# Autodesk Inventor assembly: 3.25'' Traction Wheel, Square Insert2
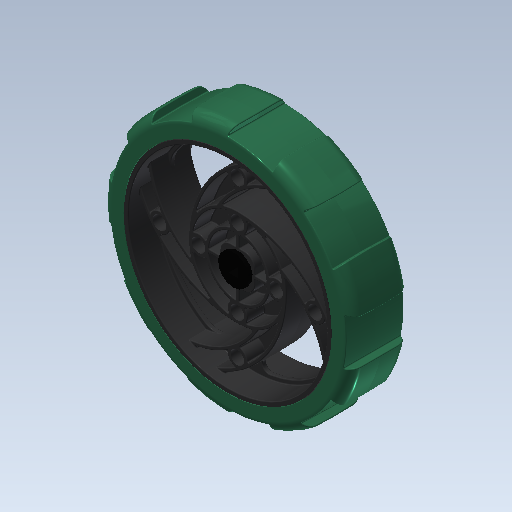
[picture p0: Inventor's stored thumbnail of the model, 512x512]
Saved by Autodesk Inventor 2020 (Build 240168000, 168)
## iProperties
Created: 2014-08-29
Document SubType Name: Assembly
Designer: Jordan Kiesel
Vendor: VEX Robotics, Inc.
Mass: 57.114 g
Surface Area: 417.458 cm^2
Volume: 47.1689 cm^3
Density: 1.21084 g/cm^3
Part Number: 3.25'' Traction Wheel, Square Insert2
Company: Bots 'n' Stuff
Author: Jordan Kiesel
Title: 3.25" Traction Wheel, Square Insert
## Documents named in this file (3)
- D:\Robotics\CAD\2018 BNS-VRC-SID Library\Motion\Wheels _ Rollers\3.25_ Traction Wheel, Square Insert.iam
- D:\Robotics\CAD\2018 BNS-VRC-SID Library\Motion\Wheels _ Rollers\Reference Parts\3.25_ Traction Wheels\3.25_ Traction Wheel.iam
- D:\Robotics\CAD\2018 BNS-VRC-SID Library\Motion\Reference Parts\High Strength Square Gear Insert.ipt
## Components (3 placed, 2 different names)
1. 3.25_ Traction Wheel:1 [sub-assembly] — Mate:1, Mate:2, Mate:3, Mate:4, Mate:5, Mate:6
2. High Strength Square Gear Insert:1 — Mate:1, Mate:2, Mate:3
3. High Strength Square Gear Insert:2 — Mate:4, Mate:5, Mate:6
## Relationships (6: Mate 6)
- Mate:1 (0.0254 mm): 3.25_ Traction Wheel:1 ↔ High Strength Square Gear Insert:1
- Mate:2 (0.0254 mm): 3.25_ Traction Wheel:1 ↔ High Strength Square Gear Insert:1
- Mate:3: 3.25_ Traction Wheel:1 ↔ High Strength Square Gear Insert:1
- Mate:4 (0.0254 mm): 3.25_ Traction Wheel:1 ↔ High Strength Square Gear Insert:2
- Mate:5 (0.0254 mm): 3.25_ Traction Wheel:1 ↔ High Strength Square Gear Insert:2
- Mate:6: 3.25_ Traction Wheel:1 ↔ High Strength Square Gear Insert:2
